# Autodesk Inventor assembly: 100-10-FRAME-CHASSIS-ASM-01
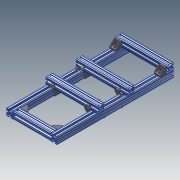
[picture p0: Inventor's stored thumbnail of the model, 180x180]
Saved by Autodesk Inventor 2018.2 (Build 222227000, 227)
## iProperties
Manager: feesmrt
Company: FRANC0R
Created: 2017-12-16
Part Number: 100-10-FRAME-CHASSIS-ASM-01
Material: Generisch
Document SubType Name: Assembly
Designer: feesmrt
Project: Rescue Robot
Cost Center: -
Description: Baseframe ASM
Engineer: feesmrt
Authority: feesmrt
Stock Number: 100-10-FRAME-CHASSIS-ASM-01
Author: feesmrt
Title: Baseframe ASM
Subject: Rescue Robot
Revision Number: 1
## Documents named in this file (9)
- D:\Programmierung\FRANC0R\CAD\02-Rocker-Bogie-Robot\100-CHASSIS\10-FRAME\100-10-FRAME-CHASSIS-ASM-01.iam
- D:\Programmierung\FRANC0R\CAD\02-Rocker-Bogie-Robot\100-CHASSIS\10-FRAME\100-10-FRAME-PROFILE-LENGTH-01.ipt
- D:\Programmierung\FRANC0R\CAD\02-Rocker-Bogie-Robot\100-CHASSIS\10-FRAME\100-10-FRAME-PROFILE-WIDTH-01.ipt
- D:\Programmierung\FRANC0R\CAD\02-Rocker-Bogie-Robot\100-CHASSIS\10-FRAME\100-10-FRAME-PROFILE-WIDTH-02.ipt
- D:\Programmierung\FRANC0R\CAD\02-Rocker-Bogie-Robot\100-CHASSIS\10-FRAME\100-10-FRAME-PROFILE-ROCKER-CONNECTOR.ipt
- D:\Programmierung\FRANC0R\CAD\02-Rocker-Bogie-Robot\900-COMPONENTS\900-50-PROFILES\900-50-PROFILES-ANGLE-CONN-30x30-02.iam
- D:\Programmierung\FRANC0R\CAD\02-Rocker-Bogie-Robot\900-COMPONENTS\900-50-PROFILES\900-50-PROFILES-ANGLE-CONN-30x30-01.iam
- D:\Programmierung\FRANC0R\CAD\02-Rocker-Bogie-Robot\100-CHASSIS\10-FRAME\100-10-FRAME-ROCKER-SCREW-01.iam
- D:\Programmierung\FRANC0R\CAD\02-Rocker-Bogie-Robot\100-CHASSIS\Chassis-Dimensions.xlsx
## Components (22 placed, 7 different names)
1. 100-10-FRAME-PROFILE-LENGTH-01:1 — Passend:1, Passend:4, Passend:6, Passend:19, Passend:23, Passend:27, Passend:34, Fluchtend:11, Passend:47, Passend:48, Passend:49, Passend:50
2. 100-10-FRAME-PROFILE-LENGTH-01:2 — Passend:2, Passend:3, Passend:5, Passend:21, Passend:25, Passend:29, Passend:31, Passend:43, Passend:44, Passend:45, Passend:46
3. 100-10-FRAME-PROFILE-WIDTH-01:2 — Passend:10, Passend:11, Passend:12, Passend:32, Fluchtend:10, Passend:33
4. 100-10-FRAME-PROFILE-WIDTH-02:1 — Passend:13, Passend:14, Fluchtend:1, Passend:20, Fluchtend:4, Passend:22, Fluchtend:5
5. 100-10-FRAME-PROFILE-ROCKER-CONNECTOR:1 — Passend:15, Passend:17, Fluchtend:3, Passend:24, Fluchtend:6, Passend:26, Fluchtend:7, Passend:39, Passend:40, Passend:41, Passend:42
6. 100-10-FRAME-PROFILE-ROCKER-CONNECTOR:2 — Passend:16, Passend:18, Fluchtend:2, Passend:28, Fluchtend:8, Passend:30, Fluchtend:9, Passend:35, Passend:36, Passend:37, Passend:38
7. 900-50-PROFILES-ANGLE-CONN-30x30-02:1 [sub-assembly] — Passend:19, Passend:20, Fluchtend:4
8. 900-50-PROFILES-ANGLE-CONN-30x30-02:2 [sub-assembly] — Passend:21, Passend:22, Fluchtend:5
9. 900-50-PROFILES-ANGLE-CONN-30x30-02:3 [sub-assembly] — Passend:23, Passend:24, Fluchtend:6
10. 900-50-PROFILES-ANGLE-CONN-30x30-02:4 [sub-assembly] — Passend:25, Passend:26, Fluchtend:7
11. 900-50-PROFILES-ANGLE-CONN-30x30-02:5 [sub-assembly] — Passend:27, Passend:28, Fluchtend:8
12. 900-50-PROFILES-ANGLE-CONN-30x30-02:6 [sub-assembly] — Passend:29, Passend:30, Fluchtend:9
13. 900-50-PROFILES-ANGLE-CONN-30x30-01:1 [sub-assembly] — Passend:31, Passend:32, Fluchtend:10
14. 900-50-PROFILES-ANGLE-CONN-30x30-01:2 [sub-assembly] — Passend:33, Passend:34, Fluchtend:11
15. 100-10-FRAME-ROCKER-SCREW-01:1 [sub-assembly] — Passend:35, Passend:36
16. 100-10-FRAME-ROCKER-SCREW-01:2 [sub-assembly] — Passend:37, Passend:38
17. 100-10-FRAME-ROCKER-SCREW-01:3 [sub-assembly] — Passend:39, Passend:40
18. 100-10-FRAME-ROCKER-SCREW-01:4 [sub-assembly] — Passend:41, Passend:42
19. 100-10-FRAME-ROCKER-SCREW-01:5 [sub-assembly] — Passend:43, Passend:44
20. 100-10-FRAME-ROCKER-SCREW-01:6 [sub-assembly] — Passend:49, Passend:50
21. 100-10-FRAME-ROCKER-SCREW-01:7 [sub-assembly] — Passend:47, Passend:48
22. 100-10-FRAME-ROCKER-SCREW-01:8 [sub-assembly] — Passend:45, Passend:46
## Relationships (58: Mate 47, Flush 11)
- Passend:1 [Mate]: 100-10-FRAME-PROFILE-LENGTH-01:1
- Passend:2 [Mate]: 100-10-FRAME-PROFILE-LENGTH-01:2
- Passend:3 [Mate]: 100-10-FRAME-PROFILE-LENGTH-01:2
- Passend:4 [Mate]: 100-10-FRAME-PROFILE-LENGTH-01:1
- Passend:5 [Mate] (-95 mm): 100-10-FRAME-PROFILE-LENGTH-01:2
- Passend:6 [Mate] (95 mm): 100-10-FRAME-PROFILE-LENGTH-01:1
- Passend:10 [Mate]: 100-10-FRAME-PROFILE-WIDTH-01:2
- Passend:11 [Mate]: 100-10-FRAME-PROFILE-WIDTH-01:2
- Passend:12 [Mate] (-235 mm): 100-10-FRAME-PROFILE-WIDTH-01:2
- Passend:13 [Mate] (30 mm): 100-10-FRAME-PROFILE-WIDTH-02:1
- Passend:14 [Mate]: 100-10-FRAME-PROFILE-WIDTH-02:1
- Fluchtend:1 [Flush] (235 mm): 100-10-FRAME-PROFILE-WIDTH-02:1
- Passend:15 [Mate] (30 mm): 100-10-FRAME-PROFILE-ROCKER-CONNECTOR:1
- Passend:16 [Mate] (30 mm): 100-10-FRAME-PROFILE-ROCKER-CONNECTOR:2
- Passend:17 [Mate]: 100-10-FRAME-PROFILE-ROCKER-CONNECTOR:1
- Passend:18 [Mate]: 100-10-FRAME-PROFILE-ROCKER-CONNECTOR:2
- Fluchtend:2 [Flush] (65 mm): 100-10-FRAME-PROFILE-ROCKER-CONNECTOR:2
- Fluchtend:3 [Flush] (-65 mm): 100-10-FRAME-PROFILE-ROCKER-CONNECTOR:1
- Passend:19 [Mate]: 100-10-FRAME-PROFILE-LENGTH-01:1 ↔ 900-50-PROFILES-ANGLE-CONN-30x30-02:1
- Passend:20 [Mate]: 100-10-FRAME-PROFILE-WIDTH-02:1 ↔ 900-50-PROFILES-ANGLE-CONN-30x30-02:1
- Fluchtend:4 [Flush]: 100-10-FRAME-PROFILE-WIDTH-02:1 ↔ 900-50-PROFILES-ANGLE-CONN-30x30-02:1
- Passend:21 [Mate]: 100-10-FRAME-PROFILE-LENGTH-01:2 ↔ 900-50-PROFILES-ANGLE-CONN-30x30-02:2
- Passend:22 [Mate]: 100-10-FRAME-PROFILE-WIDTH-02:1 ↔ 900-50-PROFILES-ANGLE-CONN-30x30-02:2
- Fluchtend:5 [Flush]: 100-10-FRAME-PROFILE-WIDTH-02:1 ↔ 900-50-PROFILES-ANGLE-CONN-30x30-02:2
- Passend:23 [Mate]: 100-10-FRAME-PROFILE-LENGTH-01:1 ↔ 900-50-PROFILES-ANGLE-CONN-30x30-02:3
- Passend:24 [Mate]: 100-10-FRAME-PROFILE-ROCKER-CONNECTOR:1 ↔ 900-50-PROFILES-ANGLE-CONN-30x30-02:3
- Fluchtend:6 [Flush]: 100-10-FRAME-PROFILE-ROCKER-CONNECTOR:1 ↔ 900-50-PROFILES-ANGLE-CONN-30x30-02:3
- Passend:25 [Mate]: 100-10-FRAME-PROFILE-LENGTH-01:2 ↔ 900-50-PROFILES-ANGLE-CONN-30x30-02:4
- Passend:26 [Mate]: 100-10-FRAME-PROFILE-ROCKER-CONNECTOR:1 ↔ 900-50-PROFILES-ANGLE-CONN-30x30-02:4
- Fluchtend:7 [Flush]: 100-10-FRAME-PROFILE-ROCKER-CONNECTOR:1 ↔ 900-50-PROFILES-ANGLE-CONN-30x30-02:4
- Passend:27 [Mate]: 100-10-FRAME-PROFILE-LENGTH-01:1 ↔ 900-50-PROFILES-ANGLE-CONN-30x30-02:5
- Passend:28 [Mate]: 100-10-FRAME-PROFILE-ROCKER-CONNECTOR:2 ↔ 900-50-PROFILES-ANGLE-CONN-30x30-02:5
- Fluchtend:8 [Flush]: 100-10-FRAME-PROFILE-ROCKER-CONNECTOR:2 ↔ 900-50-PROFILES-ANGLE-CONN-30x30-02:5
- Passend:29 [Mate]: 100-10-FRAME-PROFILE-LENGTH-01:2 ↔ 900-50-PROFILES-ANGLE-CONN-30x30-02:6
- Passend:30 [Mate]: 100-10-FRAME-PROFILE-ROCKER-CONNECTOR:2 ↔ 900-50-PROFILES-ANGLE-CONN-30x30-02:6
- Fluchtend:9 [Flush]: 100-10-FRAME-PROFILE-ROCKER-CONNECTOR:2 ↔ 900-50-PROFILES-ANGLE-CONN-30x30-02:6
- Passend:31 [Mate]: 100-10-FRAME-PROFILE-LENGTH-01:2 ↔ 900-50-PROFILES-ANGLE-CONN-30x30-01:1
- Passend:32 [Mate]: 100-10-FRAME-PROFILE-WIDTH-01:2 ↔ 900-50-PROFILES-ANGLE-CONN-30x30-01:1
- Fluchtend:10 [Flush]: 100-10-FRAME-PROFILE-WIDTH-01:2 ↔ 900-50-PROFILES-ANGLE-CONN-30x30-01:1
- Passend:33 [Mate]: 100-10-FRAME-PROFILE-WIDTH-01:2 ↔ 900-50-PROFILES-ANGLE-CONN-30x30-01:2
- Passend:34 [Mate]: 100-10-FRAME-PROFILE-LENGTH-01:1 ↔ 900-50-PROFILES-ANGLE-CONN-30x30-01:2
- Fluchtend:11 [Flush]: 100-10-FRAME-PROFILE-LENGTH-01:1 ↔ 900-50-PROFILES-ANGLE-CONN-30x30-01:2
- Passend:35 [Mate]: 100-10-FRAME-PROFILE-ROCKER-CONNECTOR:2 ↔ 100-10-FRAME-ROCKER-SCREW-01:1
- Passend:36 [Mate]: 100-10-FRAME-PROFILE-ROCKER-CONNECTOR:2 ↔ 100-10-FRAME-ROCKER-SCREW-01:1
- Passend:37 [Mate]: 100-10-FRAME-PROFILE-ROCKER-CONNECTOR:2 ↔ 100-10-FRAME-ROCKER-SCREW-01:2
- Passend:38 [Mate]: 100-10-FRAME-PROFILE-ROCKER-CONNECTOR:2 ↔ 100-10-FRAME-ROCKER-SCREW-01:2
- Passend:39 [Mate]: 100-10-FRAME-PROFILE-ROCKER-CONNECTOR:1 ↔ 100-10-FRAME-ROCKER-SCREW-01:3
- Passend:40 [Mate]: 100-10-FRAME-PROFILE-ROCKER-CONNECTOR:1 ↔ 100-10-FRAME-ROCKER-SCREW-01:3
- Passend:41 [Mate]: 100-10-FRAME-PROFILE-ROCKER-CONNECTOR:1 ↔ 100-10-FRAME-ROCKER-SCREW-01:4
- Passend:42 [Mate]: 100-10-FRAME-PROFILE-ROCKER-CONNECTOR:1 ↔ 100-10-FRAME-ROCKER-SCREW-01:4
- Passend:43 [Mate]: 100-10-FRAME-PROFILE-LENGTH-01:2 ↔ 100-10-FRAME-ROCKER-SCREW-01:5
- Passend:44 [Mate]: 100-10-FRAME-PROFILE-LENGTH-01:2 ↔ 100-10-FRAME-ROCKER-SCREW-01:5
- Passend:45 [Mate]: 100-10-FRAME-PROFILE-LENGTH-01:2 ↔ 100-10-FRAME-ROCKER-SCREW-01:8
- Passend:46 [Mate]: 100-10-FRAME-PROFILE-LENGTH-01:2 ↔ 100-10-FRAME-ROCKER-SCREW-01:8
- Passend:47 [Mate]: 100-10-FRAME-PROFILE-LENGTH-01:1 ↔ 100-10-FRAME-ROCKER-SCREW-01:7
- Passend:48 [Mate]: 100-10-FRAME-PROFILE-LENGTH-01:1 ↔ 100-10-FRAME-ROCKER-SCREW-01:7
- Passend:49 [Mate]: 100-10-FRAME-PROFILE-LENGTH-01:1 ↔ 100-10-FRAME-ROCKER-SCREW-01:6
- Passend:50 [Mate]: 100-10-FRAME-PROFILE-LENGTH-01:1 ↔ 100-10-FRAME-ROCKER-SCREW-01:6
## Named parameters: Chassis_Length = 500 mm, Chassis_Width = 220 mm, Chassis_Frame_Size = 30 mm, Rocker_Bearing_Size = 100 mm, Rocker_Screw_Distance = 32.5 mm, Rocker_Screw_Distance_Bottom = 76 mm
